# Autodesk Inventor assembly: DriveChain V4
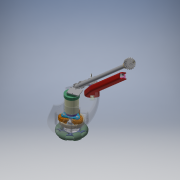
[picture p0: Inventor's stored thumbnail of the model, 180x180]
Saved by Autodesk Inventor 2019.1 (Build 231200000, 200)
## iProperties
Created: 2018-11-14
Part Number: DriveChain V4
Material: Generisch
Document SubType Name: Assembly
Designer: JochenAlt
Author: JochenAlt
## Documents named in this file (9)
- D:\Projects\Ondine\CAD\DriveChain V4.iam
- D:\Projects\Ondine\CAD\DriveChainEnclosure V4.ipt
- D:\Projects\Ondine\CAD\BushOmniWheelV3.ipt
- D:\Projects\Ondine\CAD\Leg\Worm.iam
- D:\Projects\Ondine\CAD\Leg\LegRod.iam
- D:\Projects\Ondine\CAD\Bearings\W 617_3.iam
- D:\Projects\Ondine\CAD\Leg\Leg V4.iam
- D:\Projects\Ondine\CAD\Leg\LegAxis.ipt
- D:\Projects\Ondine\CAD\PlanetaryGear2\MotorChainV4.iam
## Components (11 placed, 8 different names)
1. DriveChainEnclosure:1 — Passend:12, Passend:17, Passend:42, Passend:43, Passend:44, Passend:45, Passend:46, Passend:47, Passend:55, Winkel:1, Passend:56, Passend:58, Passend:59, Passend:60
2. BushOmniWheel:1 — Passend:12, Passend:17
3. Worm:1 [sub-assembly] — Passend:42, Passend:43, Passend:48, Passend:49, Passend:50, Drehung:1
4. LegRod:1 [sub-assembly] — Passend:44, Passend:45, Passend:51, Passend:52, Passend:53, Drehung:1
5. W 617_3:1 [sub-assembly] — Passend:46, Passend:51
6. W 617_3:2 [sub-assembly] — Passend:47, Passend:50
7. W 617_3:3 [sub-assembly] — Passend:48, Passend:49
8. W 617_3:4 [sub-assembly] — Passend:52, Passend:53
9. Leg V4:1 [sub-assembly] — Passend:55, Winkel:1, Passend:56, Passend:57
10. LegAxis:1 — Passend:57
11. MotorChainV4:1 [sub-assembly] — Passend:58, Passend:59, Passend:60
## Relationships (22: Mate 20, RelateRotation 1, Angle 1)
- Passend:12 [Mate]: DriveChainEnclosure:1 ↔ BushOmniWheel:1
- Passend:17 [Mate]: DriveChainEnclosure:1 ↔ BushOmniWheel:1
- Passend:42 [Mate]: DriveChainEnclosure:1 ↔ Worm:1
- Passend:43 [Mate]: DriveChainEnclosure:1 ↔ Worm:1
- Passend:44 [Mate]: DriveChainEnclosure:1 ↔ LegRod:1
- Passend:45 [Mate]: DriveChainEnclosure:1 ↔ LegRod:1
- Passend:46 [Mate]: DriveChainEnclosure:1 ↔ W 617_3:1
- Passend:47 [Mate]: DriveChainEnclosure:1 ↔ W 617_3:2
- Passend:48 [Mate]: Worm:1 ↔ W 617_3:3
- Passend:49 [Mate]: Worm:1 ↔ W 617_3:3
- Passend:50 [Mate]: Worm:1 ↔ W 617_3:2
- Passend:51 [Mate]: LegRod:1 ↔ W 617_3:1
- Passend:52 [Mate]: LegRod:1 ↔ W 617_3:4
- Passend:53 [Mate]: LegRod:1 ↔ W 617_3:4
- Drehung:1 [RelateRotation] (1 ul): Worm:1 ↔ LegRod:1
- Passend:55 [Mate]: DriveChainEnclosure:1 ↔ Leg V4:1
- Winkel:1 [Angle] (180 deg): DriveChainEnclosure:1 ↔ Leg V4:1
- Passend:56 [Mate]: DriveChainEnclosure:1 ↔ Leg V4:1
- Passend:57 [Mate]: Leg V4:1 ↔ LegAxis:1
- Passend:58 [Mate]: DriveChainEnclosure:1 ↔ MotorChainV4:1
- Passend:59 [Mate]: DriveChainEnclosure:1 ↔ MotorChainV4:1
- Passend:60 [Mate] (0.2 mm): DriveChainEnclosure:1 ↔ MotorChainV4:1
